# Autodesk Inventor assembly: Gears - Complete
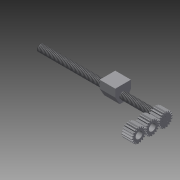
[picture p0: Inventor's stored thumbnail of the model, 180x180]
Saved by Autodesk Inventor 2014 (Build 180170000, 170)
## iProperties
Created: 2014-03-13
Part Number: Gears - Complete
Document SubType Name: Assembly
Designer: John
Author: John
## Documents named in this file (4)
- C:\File Storage\Lynda\Inventor Essentials\Ex_Files_Autodesk_Inv_Ess\Exercise Files\15_Using constraints to position parts\15_06\Gears - Complete.iam
- C:\File Storage\Lynda\Inventor Essentials\Ex_Files_Autodesk_Inv_Ess\Exercise Files\15_Using constraints to position parts\15_06\Gear.ipt
- C:\File Storage\Lynda\Inventor Essentials\Ex_Files_Autodesk_Inv_Ess\Exercise Files\15_Using constraints to position parts\15_06\Threaded Shaft.ipt
- C:\File Storage\Lynda\Inventor Essentials\Ex_Files_Autodesk_Inv_Ess\Exercise Files\15_Using constraints to position parts\15_06\Linear Stage.ipt
## Components (5 placed, 3 different names)
1. Gear:1 — Mate:1, Mate:2, Flush:1, Flush:2, Angle:2 - DRIVE, Rotation:1, Rotation:2
2. Gear:2 — Flush:1, Mate:3, Mate:5, Rotation:1
3. Gear:3 — Flush:2, Mate:4, Mate:6, Insert:1, Mate:7, Rotation:2
4. Threaded Shaft:1 — Insert:1, Mate:7, Mate:8, Rotation/Translation:1
5. Linear Stage:1 — Mate:8, Angle:1, Rotation/Translation:1
## Relationships (16: Mate 8, Flush 2, Angle 2, RelateRotation 2, Insert 1, RelateRotateTranslate 1)
- Mate:1: Gear:1
- Mate:2: Gear:1
- Flush:1: Gear:1 ↔ Gear:2
- Flush:2: Gear:1 ↔ Gear:3
- Mate:3: Gear:2
- Mate:4: Gear:3
- Mate:5 (16.1925 mm): Gear:2
- Mate:6 (-16.1925 mm): Gear:3
- Insert:1: Gear:3 ↔ Threaded Shaft:1
- Mate:7: Gear:3 ↔ Threaded Shaft:1
- Mate:8: Threaded Shaft:1 ↔ Linear Stage:1
- Angle:1 (0 deg): Linear Stage:1
- Angle:2 - DRIVE (0 deg): Gear:1
- Rotation:1 [RelateRotation] (1 ul): Gear:1 ↔ Gear:2
- Rotation:2 [RelateRotation] (1 ul): Gear:1 ↔ Gear:3
- Rotation/Translation:1 [RelateRotateTranslate] (12.7 mm): Threaded Shaft:1 ↔ Linear Stage:1
